# Autodesk Inventor assembly: BlankGearbox
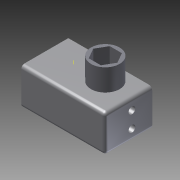
[picture p0: Inventor's stored thumbnail of the model, 180x180]
Saved by Autodesk Inventor 2012 (Build 160160000, 160)
## iProperties
Created: 2011-10-24
Part Number: BlankGearbox
Document SubType Name: Assembly
Designer: KuttaA
Author: KuttaA
## Documents named in this file (6)
- C:\Users\KuttaA\Dropbox\Hexapod Research\Leg Design\Other Parts\Intermediary Gear Box\BlankGearbox.iam
- C:\Users\KuttaA\Dropbox\Hexapod Research\Leg Design\Other Parts\Intermediary Gear Box\GearboxWallOutput.ipt
- C:\Users\KuttaA\Dropbox\Hexapod Research\Leg Design\Other Parts\Intermediary Gear Box\BlankSmallGearOutput.ipt
- C:\Users\KuttaA\Dropbox\Hexapod Research\Leg Design\Other Parts\Intermediary Gear Box\BlankLargeGearMotorInput.ipt
- C:\Users\KuttaA\Dropbox\Hexapod Research\Leg Design\Other Parts\Intermediary Gear Box\BlankGearLargeAndSmall.ipt
- C:\Users\KuttaA\Dropbox\Hexapod Research\Leg Design\Other Parts\Intermediary Gear Box\LargeSmallGearAxis.ipt
## Components (5 placed, 5 different names)
1. GearboxWallOutput:1 — Mate:1, Mate:2, Mate:3, Mate:4, Mate:7, Mate:8, Mate:9
2. BlankSmallGearOutput:1 — Mate:1, Mate:2
3. BlankLargeGearMotorInput:1 — Mate:3, Mate:4
4. BlankGearLargeAndSmall:1 — Mate:5, Mate:6
5. LargeSmallGearAxis:1 — Mate:5, Mate:6, Mate:7, Mate:8, Mate:9
## Relationships (9: Mate 9)
- Mate:1 (0.3 mm): GearboxWallOutput:1 ↔ BlankSmallGearOutput:1
- Mate:2: GearboxWallOutput:1 ↔ BlankSmallGearOutput:1
- Mate:3 (0.3 mm): GearboxWallOutput:1 ↔ BlankLargeGearMotorInput:1
- Mate:4: GearboxWallOutput:1 ↔ BlankLargeGearMotorInput:1
- Mate:5: BlankGearLargeAndSmall:1 ↔ LargeSmallGearAxis:1
- Mate:6 (0.3 mm): BlankGearLargeAndSmall:1 ↔ LargeSmallGearAxis:1
- Mate:7 (0.3 mm): GearboxWallOutput:1 ↔ LargeSmallGearAxis:1
- Mate:8 (1 mm): GearboxWallOutput:1 ↔ LargeSmallGearAxis:1
- Mate:9 (0.3 mm): GearboxWallOutput:1 ↔ LargeSmallGearAxis:1
